# Autodesk Inventor assembly: mainAssy
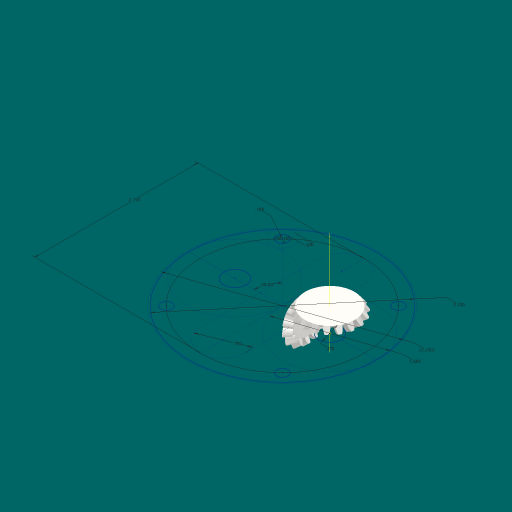
[picture p0: Inventor's stored thumbnail of the model, 512x512]
Saved by Autodesk Inventor 2023.1 (Build 271208000, 208)
## iProperties
Created: 2022-10-10
Part Number: mainAssy
Document SubType Name: Assembly
Designer: zac-h
Author: zac-h
## Documents named in this file (3)
- C:\Users\zac-h\Documents\CAD\guardSwerve4\mainAssy.iam
- C:\Users\zac-h\Documents\CAD\guardSwerve4\carriage.ipt
- C:\Users\zac-h\Documents\CAD\guardSwerve4\mainAssy\Design Accelerator\Bevel Gears1.iam
## Components (2 placed, 2 different names)
1. Bevel Gears:1 [sub-assembly] — Mate:1, Angle:1, Mate:2
2. carriage:1
## Relationships (3: Mate 2, Angle 1)
- Mate:1: Bevel Gears:1
- Angle:1 (0 deg): Bevel Gears:1
- Mate:2: Bevel Gears:1
